# Autodesk Inventor assembly: Clamp(maxOpening40mm)-sample
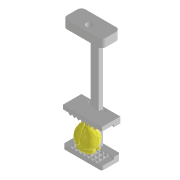
[picture p0: Inventor's stored thumbnail of the model, 180x180]
Saved by Autodesk Inventor 2021 (Build 250183000, 183)
## iProperties
Created: 2023-02-13
Part Number: Clamp(maxOpening40mm)-sample
Document SubType Name: Assembly
Designer: nvladi
Author: nvladi
## Documents named in this file (4)
- C:\Users\Public\GitHub-public\benchtop-hardware\Benchtop\CAD-model-Inventor2021\mesoSPIM\sample_handling\assemblies\Clamp(maxOpening40mm)-sample.iam
- C:\Users\Public\GitHub-public\benchtop-hardware\Benchtop\CAD-model-Inventor2021\mesoSPIM\sample_handling\sample-holders\Clamp-part1-Base9x19mm-maxSample40mm.ipt
- C:\Users\Public\GitHub-public\benchtop-hardware\Benchtop\CAD-model-Inventor2021\mesoSPIM\sample_handling\sample-holders\Clamp-part2(moving)-Base9x19mm_100912(01)_C.ipt
- C:\Users\Public\GitHub-public\benchtop-hardware\Benchtop\CAD-model-Inventor2021\library\samples\mousebrain2.ipt
## Components (3 placed, 3 different names)
1. Clamp-part1-Base9x19mm-maxSample40mm:1 — Mate:1, Mate:2
2. Clamp-part2(moving)-Base9x19mm_100912(01)_C:1 — Mate:1, Mate:2
3. mousebrain2:1
## Relationships (2: Mate 2)
- Mate:1: Clamp-part1-Base9x19mm-maxSample40mm:1 ↔ Clamp-part2(moving)-Base9x19mm_100912(01)_C:1
- Mate:2: Clamp-part1-Base9x19mm-maxSample40mm:1 ↔ Clamp-part2(moving)-Base9x19mm_100912(01)_C:1
